# Autodesk Inventor assembly: Robot3
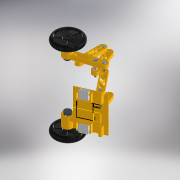
[picture p0: Inventor's stored thumbnail of the model, 180x180]
Saved by Autodesk Inventor 2021 (Build 250183000, 183)
## iProperties
Created: 2024-02-25
Part Number: Robot3
Document SubType Name: Assembly
Designer: Martin
Author: Martin
## Documents named in this file (20)
- C:\Users\ASUS\OneDrive - Universidad de Antioquia\2024-1\Robótica\Proyecto\CAD\Robot3.iam
- C:\Users\ASUS\OneDrive - Universidad de Antioquia\2024-1\Robótica\Proyecto\CAD\op1\EslabonCodoTrasero.ipt
- C:\Users\ASUS\OneDrive - Universidad de Antioquia\2024-1\Robótica\Proyecto\CAD\op1\EslabonRodillaCadera.ipt
- C:\Users\ASUS\OneDrive - Universidad de Antioquia\2024-1\Robótica\Proyecto\CAD\op1\EslabonRuedaRodilla.ipt
- C:\Users\ASUS\Documents\Inventor\Content Center Files\R2021\en-US\DIN 625 SKF(3)\DIN 625 SKF - SKF 608-RSL.ipt
- C:\Users\ASUS\OneDrive - Universidad de Antioquia\2024-1\Robótica\Proyecto\CAD\op1\Buje.ipt
- C:\Users\ASUS\OneDrive - Universidad de Antioquia\2024-1\Robótica\Proyecto\CAD\Llanta.ipt
- C:\Users\ASUS\OneDrive - Universidad de Antioquia\2024-1\Robótica\Proyecto\CAD\Resorte.ipt
- C:\Users\ASUS\OneDrive - Universidad de Antioquia\2024-1\Robótica\Proyecto\CAD\Carcasa.ipt
- C:\Users\ASUS\Documents\Inventor\Content Center Files\R2021\en-US\AS 1110\AS 1110 - M8 x 80.ipt
- C:\Users\ASUS\OneDrive - Universidad de Antioquia\2024-1\Robótica\Proyecto\CAD\Servo.ipt
- C:\Users\ASUS\OneDrive - Universidad de Antioquia\2024-1\Robótica\Proyecto\CAD\37d-gearmotor-19-30-encoder.ipt
- C:\Users\ASUS\OneDrive - Universidad de Antioquia\2024-1\Robótica\Proyecto\CAD\op1\EslabonCodoTrasero_MIR.ipt
- C:\Users\ASUS\OneDrive - Universidad de Antioquia\2024-1\Robótica\Proyecto\CAD\op1\EslabonRodillaCadera_MIR.ipt
- C:\Users\ASUS\OneDrive - Universidad de Antioquia\2024-1\Robótica\Proyecto\CAD\op1\EslabonRuedaRodilla_MIR.ipt
- C:\Users\ASUS\OneDrive - Universidad de Antioquia\2024-1\Robótica\Proyecto\CAD\op1\Buje_MIR.ipt
- C:\Users\ASUS\OneDrive - Universidad de Antioquia\2024-1\Robótica\Proyecto\CAD\Llanta_MIR1.ipt
- C:\Users\ASUS\OneDrive - Universidad de Antioquia\2024-1\Robótica\Proyecto\CAD\Resorte_MIR1.ipt
- C:\Users\ASUS\OneDrive - Universidad de Antioquia\2024-1\Robótica\Proyecto\CAD\Servo_MIR1.ipt
- C:\Users\ASUS\OneDrive - Universidad de Antioquia\2024-1\Robótica\Proyecto\CAD\37d-gearmotor-19-30-encoder_MIR.ipt
## Components (37 placed, 19 different names)
1. EslabonCodoTrasero:1 — Mate:4, Mate:6, Flush:1, Mate:11, Mate:12, Mate:32, Mate:33, Mate:46, Mate:47
2. EslabonRodillaCadera:1 — Mate:2, Mate:3, Mate:13, Mate:14, Mate:22, Mate:25, Mate:53
3. EslabonRuedaRodilla:1 — Mate:2, Mate:3, Mate:4, Mate:7, Mate:8, Mate:9, Mate:10, Mate:23, Mate:24, Mate:30, Mate:54, Mate:55
4. DIN 625 SKF- with one low-friction seal SKF 608-RSL:1 — Mate:6, Flush:1
5. DIN 625 SKF- with one low-friction seal SKF 608-RSL:2 — Mate:9, Mate:10, Mate:45
6. DIN 625 SKF- with one low-friction seal SKF 608-RSL:3 — Mate:11, Mate:12
7. DIN 625 SKF- with one low-friction seal SKF 608-RSL:4 — Mate:7, Mate:8, Mate:28, Mate:29
8. DIN 625 SKF- with one low-friction seal SKF 608-RSL:5 — Mate:13, Mate:14, Mate:31
9. Buje:1 — Flush:2
10. Llanta:1 — Flush:2
11. Resorte:1 — Mate:22, Mate:25
12. DIN 625 SKF- with one low-friction seal SKF 608-RSL:6 — Mate:23, Mate:24
13. Carcasa:1 — Mate:47, Mate:48, Mate:49, Mate:51, Mate:52
14. AS 1110 - Metric M8 x 80:1 — Mate:28, Mate:29, Mate:46
15. DIN 625 SKF- with one low-friction seal SKF 608-RSL:7 — Mate:30
16. AS 1110 - Metric M8 x 80:2 — Mate:31, Mate:45
17. AS 1110 - Metric M8 x 80:3 — Mate:32, Mate:33, Mate:48
18. Servo:1 — Mate:49, Mate:51, Mate:52, Mate:53
19. 37d-gearmotor-19-30-encoder:1 — Mate:54, Mate:55
20. EslabonCodoTrasero_MIR:1 — Mate:56, Flush:3, Mate:59, Mate:62, Mate:63, Mate:72, Mate:78, Mate:79
21. EslabonRodillaCadera_MIR:1 — Mate:57, Mate:58, Mate:66, Mate:67, Mate:68, Mate:69, Mate:80
22. EslabonRuedaRodilla_MIR:1 — Mate:56, Mate:57, Mate:58, Mate:60, Mate:61, Mate:64, Mate:65, Mate:70, Mate:71, Mate:75, Mate:81, Mate:82
23. DIN 625 SKF- with one low-friction seal SKF 608-RSL:8 — Flush:3, Mate:59
24. DIN 625 SKF- with one low-friction seal SKF 608-RSL:9 — Mate:60, Mate:61, Mate:76
25. DIN 625 SKF- with one low-friction seal SKF 608-RSL:10 — Mate:62, Mate:63
26. DIN 625 SKF- with one low-friction seal SKF 608-RSL:11 — Mate:64, Mate:65, Mate:73, Mate:74
27. DIN 625 SKF- with one low-friction seal SKF 608-RSL:12 — Mate:66, Mate:67, Mate:77
28. Buje_MIR:1 — Flush:4
29. Llanta_MIR1:1 — Flush:4
30. Resorte_MIR1:1 — Mate:68, Mate:69
31. DIN 625 SKF- with one low-friction seal SKF 608-RSL:13 — Mate:70, Mate:71
32. AS 1110 - Metric M8 x 80:4 — Mate:72, Mate:73, Mate:74
33. DIN 625 SKF- with one low-friction seal SKF 608-RSL:14 — Mate:75
34. AS 1110 - Metric M8 x 80:5 — Mate:76, Mate:77
35. AS 1110 - Metric M8 x 80:6 — Mate:78, Mate:79
36. Servo_MIR1:1 — Mate:80
37. 37d-gearmotor-19-30-encoder_MIR:1 — Mate:81, Mate:82
## Relationships (63: Mate 59, Flush 4)
- Mate:2: EslabonRodillaCadera:1 ↔ EslabonRuedaRodilla:1
- Mate:3 (20 mm): EslabonRodillaCadera:1 ↔ EslabonRuedaRodilla:1
- Mate:4 (20 mm): EslabonCodoTrasero:1 ↔ EslabonRuedaRodilla:1
- Mate:6: EslabonCodoTrasero:1 ↔ DIN 625 SKF- with one low-friction seal SKF 608-RSL:1
- Flush:1: EslabonCodoTrasero:1 ↔ DIN 625 SKF- with one low-friction seal SKF 608-RSL:1
- Mate:7: EslabonRuedaRodilla:1 ↔ DIN 625 SKF- with one low-friction seal SKF 608-RSL:4
- Mate:8: EslabonRuedaRodilla:1 ↔ DIN 625 SKF- with one low-friction seal SKF 608-RSL:4
- Mate:9: EslabonRuedaRodilla:1 ↔ DIN 625 SKF- with one low-friction seal SKF 608-RSL:2
- Mate:10: EslabonRuedaRodilla:1 ↔ DIN 625 SKF- with one low-friction seal SKF 608-RSL:2
- Mate:11: EslabonCodoTrasero:1 ↔ DIN 625 SKF- with one low-friction seal SKF 608-RSL:3
- Mate:12: EslabonCodoTrasero:1 ↔ DIN 625 SKF- with one low-friction seal SKF 608-RSL:3
- Mate:13: EslabonRodillaCadera:1 ↔ DIN 625 SKF- with one low-friction seal SKF 608-RSL:5
- Mate:14: EslabonRodillaCadera:1 ↔ DIN 625 SKF- with one low-friction seal SKF 608-RSL:5
- Flush:2: Buje:1 ↔ Llanta:1
- Mate:22: EslabonRodillaCadera:1 ↔ Resorte:1
- Mate:23: EslabonRuedaRodilla:1 ↔ DIN 625 SKF- with one low-friction seal SKF 608-RSL:6
- Mate:24: EslabonRuedaRodilla:1 ↔ DIN 625 SKF- with one low-friction seal SKF 608-RSL:6
- Mate:25: EslabonRodillaCadera:1 ↔ Resorte:1
- Mate:28: DIN 625 SKF- with one low-friction seal SKF 608-RSL:4 ↔ AS 1110 - Metric M8 x 80:1
- Mate:29: DIN 625 SKF- with one low-friction seal SKF 608-RSL:4 ↔ AS 1110 - Metric M8 x 80:1
- Mate:30: EslabonRuedaRodilla:1 ↔ DIN 625 SKF- with one low-friction seal SKF 608-RSL:7
- Mate:31: DIN 625 SKF- with one low-friction seal SKF 608-RSL:5 ↔ AS 1110 - Metric M8 x 80:2
- Mate:32: EslabonCodoTrasero:1 ↔ AS 1110 - Metric M8 x 80:3
- Mate:33: EslabonCodoTrasero:1 ↔ AS 1110 - Metric M8 x 80:3
- Mate:45: DIN 625 SKF- with one low-friction seal SKF 608-RSL:2 ↔ AS 1110 - Metric M8 x 80:2
- Mate:46: EslabonCodoTrasero:1 ↔ AS 1110 - Metric M8 x 80:1
- Mate:47: EslabonCodoTrasero:1 ↔ Carcasa:1
- Mate:48: Carcasa:1 ↔ AS 1110 - Metric M8 x 80:3
- Mate:49: Carcasa:1 ↔ Servo:1
- Mate:51 (1 mm): Carcasa:1 ↔ Servo:1
- Mate:52: Carcasa:1 ↔ Servo:1
- Mate:53: EslabonRodillaCadera:1 ↔ Servo:1
- Mate:54: EslabonRuedaRodilla:1 ↔ 37d-gearmotor-19-30-encoder:1
- Mate:55: EslabonRuedaRodilla:1 ↔ 37d-gearmotor-19-30-encoder:1
- Mate:56 (20 mm): EslabonCodoTrasero_MIR:1 ↔ EslabonRuedaRodilla_MIR:1
- Mate:57 (20 mm): EslabonRodillaCadera_MIR:1 ↔ EslabonRuedaRodilla_MIR:1
- Mate:58: EslabonRodillaCadera_MIR:1 ↔ EslabonRuedaRodilla_MIR:1
- Flush:3: EslabonCodoTrasero_MIR:1 ↔ DIN 625 SKF- with one low-friction seal SKF 608-RSL:8
- Mate:59: EslabonCodoTrasero_MIR:1 ↔ DIN 625 SKF- with one low-friction seal SKF 608-RSL:8
- Mate:60: EslabonRuedaRodilla_MIR:1 ↔ DIN 625 SKF- with one low-friction seal SKF 608-RSL:9
- Mate:61: EslabonRuedaRodilla_MIR:1 ↔ DIN 625 SKF- with one low-friction seal SKF 608-RSL:9
- Mate:62: EslabonCodoTrasero_MIR:1 ↔ DIN 625 SKF- with one low-friction seal SKF 608-RSL:10
- Mate:63: EslabonCodoTrasero_MIR:1 ↔ DIN 625 SKF- with one low-friction seal SKF 608-RSL:10
- Mate:64: EslabonRuedaRodilla_MIR:1 ↔ DIN 625 SKF- with one low-friction seal SKF 608-RSL:11
- Mate:65: EslabonRuedaRodilla_MIR:1 ↔ DIN 625 SKF- with one low-friction seal SKF 608-RSL:11
- Mate:66: EslabonRodillaCadera_MIR:1 ↔ DIN 625 SKF- with one low-friction seal SKF 608-RSL:12
- Mate:67: EslabonRodillaCadera_MIR:1 ↔ DIN 625 SKF- with one low-friction seal SKF 608-RSL:12
- Flush:4: Buje_MIR:1 ↔ Llanta_MIR1:1
- Mate:68: EslabonRodillaCadera_MIR:1 ↔ Resorte_MIR1:1
- Mate:69: EslabonRodillaCadera_MIR:1 ↔ Resorte_MIR1:1
- Mate:70: EslabonRuedaRodilla_MIR:1 ↔ DIN 625 SKF- with one low-friction seal SKF 608-RSL:13
- Mate:71: EslabonRuedaRodilla_MIR:1 ↔ DIN 625 SKF- with one low-friction seal SKF 608-RSL:13
- Mate:72: EslabonCodoTrasero_MIR:1 ↔ AS 1110 - Metric M8 x 80:4
- Mate:73: DIN 625 SKF- with one low-friction seal SKF 608-RSL:11 ↔ AS 1110 - Metric M8 x 80:4
- Mate:74: DIN 625 SKF- with one low-friction seal SKF 608-RSL:11 ↔ AS 1110 - Metric M8 x 80:4
- Mate:75: EslabonRuedaRodilla_MIR:1 ↔ DIN 625 SKF- with one low-friction seal SKF 608-RSL:14
- Mate:76: DIN 625 SKF- with one low-friction seal SKF 608-RSL:9 ↔ AS 1110 - Metric M8 x 80:5
- Mate:77: DIN 625 SKF- with one low-friction seal SKF 608-RSL:12 ↔ AS 1110 - Metric M8 x 80:5
- Mate:78: EslabonCodoTrasero_MIR:1 ↔ AS 1110 - Metric M8 x 80:6
- Mate:79: EslabonCodoTrasero_MIR:1 ↔ AS 1110 - Metric M8 x 80:6
- Mate:80: EslabonRodillaCadera_MIR:1 ↔ Servo_MIR1:1
- Mate:81: EslabonRuedaRodilla_MIR:1 ↔ 37d-gearmotor-19-30-encoder_MIR:1
- Mate:82: EslabonRuedaRodilla_MIR:1 ↔ 37d-gearmotor-19-30-encoder_MIR:1
